# Autodesk Inventor assembly: Drive Body
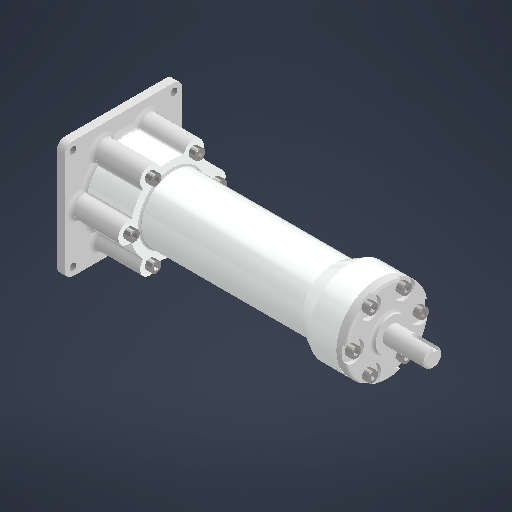
[picture p0: Inventor's stored thumbnail of the model, 512x512]
Saved by Autodesk Inventor 2026.1 (Build 301233020, 233B)
## iProperties
Created: 2025-10-14
Part Number: Drive Body
Document SubType Name: Assembly
Designer: Alexander
Author: Alexander
## Documents named in this file (11)
- C:\Users\Alexander\Documents\M&M Engineering Second year\Semester 2\Introductory Machine Design 254\Theory of Machines\Project\Part 2\Drive Body.iam
- C:\Users\Alexander\Documents\M&M Engineering Second year\Semester 2\Introductory Machine Design 254\Theory of Machines\Project\Part 2\Body.ipt
- C:\Users\Alexander\Documents\M&M Engineering Second year\Semester 2\Introductory Machine Design 254\Theory of Machines\Project\Part 2\Shaft.ipt
- C:\Users\Alexander\Documents\Inventor\Content Center Files\R2026\en-US\ISO 6194_1(2)\ISO 6194_1 - 25x47x7-Type 2.ipt
- C:\Users\Alexander\Documents\M&M Engineering Second year\Semester 2\Introductory Machine Design 254\Theory of Machines\Project\Part 2\Drive Body\Design Accelerator\Bearing2.iam
- C:\Users\Alexander\Documents\M&M Engineering Second year\Semester 2\Introductory Machine Design 254\Theory of Machines\Project\Part 2\END CAP.ipt
- C:\Users\Alexander\Documents\M&M Engineering Second year\Semester 2\Introductory Machine Design 254\Theory of Machines\Project\Part 2\Drive Body\Design Accelerator\Bearing3.iam
- C:\Users\Alexander\Documents\M&M Engineering Second year\Semester 2\Introductory Machine Design 254\Theory of Machines\Project\Part 2\BASE COVER.ipt
- C:\Users\Alexander\Documents\Inventor\Content Center Files\R2026\en-US\DIN 471(1)\DIN 471 - 25x1.2.ipt
- C:\Users\Alexander\Documents\Inventor\Content Center Files\R2026\en-US\ISO 4762(2)\ISO 4762 - M8 x 20ISO.ipt
- C:\Users\Alexander\Documents\Inventor\Content Center Files\R2026\en-US\ISO 4762(2)\ISO 4762 - M8 x 65ISO.ipt
## Components (21 placed, 9 different names)
1. Body:1 — Mate:2, Mate:14, Mate:16, Mate:17, Mate:23, Mate:24, Mate:37, Mate:38, Mate:39, Mate:40, Mate:41, Mate:42, Mate:43, Mate:44, Mate:45, Mate:46, Mate:47, Mate:48
2. Shaft:1 — Mate:2, Mate:10, Mate:11, Mate:15, Mate:18, Mate:19, Mate:22, Insert:1
3. ISO 6194/1 25x47x7-Type 2:1 — Mate:12, Mate:13
4. Bearing:1 [sub-assembly] — Mate:10, Mate:11, Mate:12, Mate:13, Mate:14
5. END CAP:1 — Mate:15, Mate:16, Mate:17, Mate:25, Mate:26, Mate:27, Mate:28, Mate:29, Mate:30, Mate:31, Mate:32, Mate:33, Mate:34, Mate:35, Mate:36
6. Bearing:2 [sub-assembly] — Mate:18, Mate:19, Mate:20, Mate:21
7. ISO 6194/1 25x47x7-Type 2:2 — Mate:20, Mate:21
8. BASE COVER:1 — Mate:22, Mate:23, Mate:24
9. DIN 471 25x1.2:1 — Insert:1
10. ISO 4762 M8 x 20:1 — Mate:25, Mate:26
11. ISO 4762 M8 x 20:2 — Mate:27, Mate:33
12. ISO 4762 M8 x 20:3 — Mate:28, Mate:34
13. ISO 4762 M8 x 20:4 — Mate:31, Mate:36
14. ISO 4762 M8 x 20:5 — Mate:30, Mate:35
15. ISO 4762 M8 x 20:6 — Mate:29, Mate:32
16. ISO 4762 M8 x 65:1 — Mate:37, Mate:47
17. ISO 4762 M8 x 65:2 — Mate:40, Mate:43
18. ISO 4762 M8 x 65:3 — Mate:38, Mate:46
19. ISO 4762 M8 x 65:4 — Mate:39, Mate:45
20. ISO 4762 M8 x 65:5 — Mate:42, Mate:48
21. ISO 4762 M8 x 65:6 — Mate:41, Mate:44
## Relationships (41: Mate 40, Insert 1)
- Mate:2: Body:1 ↔ Shaft:1
- Mate:10: Shaft:1 ↔ Bearing:1
- Mate:11: Shaft:1 ↔ Bearing:1
- Mate:12: ISO 6194/1 25x47x7-Type 2:1 ↔ Bearing:1
- Mate:13: ISO 6194/1 25x47x7-Type 2:1 ↔ Bearing:1
- Mate:14: Body:1 ↔ Bearing:1
- Mate:15: Shaft:1 ↔ END CAP:1
- Mate:16: Body:1 ↔ END CAP:1
- Mate:17: Body:1 ↔ END CAP:1
- Mate:18 (1 mm): Shaft:1 ↔ Bearing:2
- Mate:19: Shaft:1 ↔ Bearing:2
- Mate:20: Bearing:2 ↔ ISO 6194/1 25x47x7-Type 2:2
- Mate:21: Bearing:2 ↔ ISO 6194/1 25x47x7-Type 2:2
- Mate:22: Shaft:1 ↔ BASE COVER:1
- Mate:23: Body:1 ↔ BASE COVER:1
- Mate:24: Body:1 ↔ BASE COVER:1
- Insert:1: Shaft:1 ↔ DIN 471 25x1.2:1
- Mate:25: END CAP:1 ↔ ISO 4762 M8 x 20:1
- Mate:26: END CAP:1 ↔ ISO 4762 M8 x 20:1
- Mate:27: END CAP:1 ↔ ISO 4762 M8 x 20:2
- Mate:28: END CAP:1 ↔ ISO 4762 M8 x 20:3
- Mate:29: END CAP:1 ↔ ISO 4762 M8 x 20:6
- Mate:30: END CAP:1 ↔ ISO 4762 M8 x 20:5
- Mate:31: END CAP:1 ↔ ISO 4762 M8 x 20:4
- Mate:32: END CAP:1 ↔ ISO 4762 M8 x 20:6
- Mate:33: END CAP:1 ↔ ISO 4762 M8 x 20:2
- Mate:34: END CAP:1 ↔ ISO 4762 M8 x 20:3
- Mate:35: END CAP:1 ↔ ISO 4762 M8 x 20:5
- Mate:36: END CAP:1 ↔ ISO 4762 M8 x 20:4
- Mate:37: Body:1 ↔ ISO 4762 M8 x 65:1
- Mate:38: Body:1 ↔ ISO 4762 M8 x 65:3
- Mate:39: Body:1 ↔ ISO 4762 M8 x 65:4
- Mate:40: Body:1 ↔ ISO 4762 M8 x 65:2
- Mate:41: Body:1 ↔ ISO 4762 M8 x 65:6
- Mate:42: Body:1 ↔ ISO 4762 M8 x 65:5
- Mate:43: Body:1 ↔ ISO 4762 M8 x 65:2
- Mate:44: Body:1 ↔ ISO 4762 M8 x 65:6
- Mate:45: Body:1 ↔ ISO 4762 M8 x 65:4
- Mate:46: Body:1 ↔ ISO 4762 M8 x 65:3
- Mate:47: Body:1 ↔ ISO 4762 M8 x 65:1
- Mate:48: Body:1 ↔ ISO 4762 M8 x 65:5
